# Autodesk Inventor assembly: Fr.wing
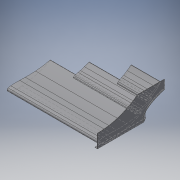
[picture p0: Inventor's stored thumbnail of the model, 180x180]
Saved by Autodesk Inventor 2018.2 (Build 222227000, 227)
## iProperties
Created: 2018-02-26
Part Number: Fr.wing
Material: 一般
Document SubType Name: Assembly
Designer: ku_sk
Author: ku_sk
## Documents named in this file (7)
- C:\Users\ku_sk\Documents\Inventor\AeroCAD2018\設計\Fr.wing\Fr.wing.iam
- C:\Users\ku_sk\Documents\Inventor\AeroCAD2018\設計\Fr.wing\parts\endplate.ipt
- C:\Users\ku_sk\Documents\Inventor\AeroCAD2018\設計\Fr.wing\parts\mainflap.ipt
- C:\Users\ku_sk\Documents\Inventor\AeroCAD2018\設計\Fr.wing\parts\subflap.ipt
- C:\Users\ku_sk\Documents\Inventor\AeroCAD2018\設計\Fr.wing\parts\subflap2.ipt
- C:\Users\ku_sk\Documents\Inventor\AeroCAD2018\設計\Fr.wing\parts\bracket.ipt
- C:\Users\ku_sk\Documents\Inventor\AeroCAD2018\設計\Fr.wing\parts\mainflapcenter.ipt
## Components (6 placed, 6 different names)
1. endplate:1 — メイト:1, メイト:2, メイト:4, メイト:5
2. mainflap:1 — メイト:2, 角度:1, メイト:6
3. subflap:2 — メイト:4, 角度:2
4. subflap2:1 — メイト:5, 角度:1, 角度:2
5. bracket:1 — メイト:6, メイト:7
6. mainflapcenter:1 — メイト:7
## Relationships (8: Mate 6, Angle 2)
- メイト:1 [Mate]: endplate:1
- メイト:2 [Mate]: endplate:1 ↔ mainflap:1
- メイト:4 [Mate]: endplate:1 ↔ subflap:2
- メイト:5 [Mate]: endplate:1 ↔ subflap2:1
- 角度:1 [Angle] (-15 deg): mainflap:1 ↔ subflap2:1
- 角度:2 [Angle] (-15 deg): subflap:2 ↔ subflap2:1
- メイト:6 [Mate]: mainflap:1 ↔ bracket:1
- メイト:7 [Mate]: bracket:1 ↔ mainflapcenter:1
